# Autodesk Inventor assembly: damascusCoverAssembly
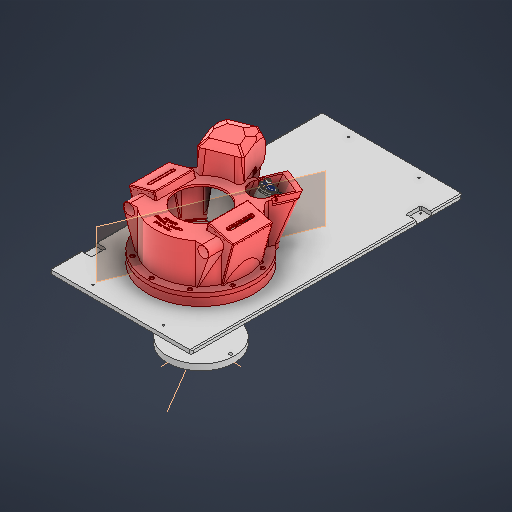
[picture p0: Inventor's stored thumbnail of the model, 512x512]
Saved by Autodesk Inventor 2026.2 (Build 302298000, 298)
## iProperties
Created: 2026-05-01
Part Number: damascusCoverAssembly
Document SubType Name: Assembly
Designer: mayhe
Author: mayhe
## Documents named in this file (10)
- C:\Users\mayhe\OneDrive\Documents\GitHub\In-situ-monitoring-of-powder-bed-fusion-additive-manufacturing\system_development\Damascus\V0.4\hardware development\damascusCoverAssembly.iam
- C:\Users\mayhe\OneDrive\Documents\GitHub\In-situ-monitoring-of-powder-bed-fusion-additive-manufacturing\system_development\Damascus\V0.4\hardware development\Parts\12mm Cover.ipt
- C:\Users\mayhe\OneDrive\Documents\GitHub\In-situ-monitoring-of-powder-bed-fusion-additive-manufacturing\system_development\Damascus\V0.4\hardware development\Parts\Build Plate with 35mm FOV Sketch.ipt
- C:\Users\mayhe\OneDrive\Documents\GitHub\In-situ-monitoring-of-powder-bed-fusion-additive-manufacturing\system_development\Damascus\V0.4\hardware development\Parts\twinHead.ipt
- C:\Users\mayhe\OneDrive\Documents\GitHub\In-situ-monitoring-of-powder-bed-fusion-additive-manufacturing\system_development\Damascus\V0.4\hardware development\Parts\sealRing.ipt
- C:\Users\mayhe\OneDrive\Documents\GitHub\In-situ-monitoring-of-powder-bed-fusion-additive-manufacturing\system_development\Damascus\V0.4\hardware development\Parts\Xi-410-Camera-with-29°-x-18°-Lens\Xi 410 Camera with 29° x.iam
- C:\Users\mayhe\OneDrive\Documents\GitHub\In-situ-monitoring-of-powder-bed-fusion-additive-manufacturing\system_development\Damascus\V0.4\hardware development\Parts\Optical Camera\Camera with 35mm.iam
- C:\Users\mayhe\OneDrive\Documents\GitHub\In-situ-monitoring-of-powder-bed-fusion-additive-manufacturing\system_development\Damascus\V0.4\hardware development\Parts\New Thermal Lid.ipt
- C:\Users\mayhe\OneDrive\Documents\GitHub\In-situ-monitoring-of-powder-bed-fusion-additive-manufacturing\system_development\Damascus\V0.4\hardware development\Parts\Antireflective Glass.ipt
- C:\Users\mayhe\OneDrive\Documents\GitHub\In-situ-monitoring-of-powder-bed-fusion-additive-manufacturing\system_development\Damascus\V0.4\hardware development\Parts\opticalLid.ipt
## Components (9 placed, 9 different names)
1. 12mm Cover:1 — Rotational:1, Rotational:2
2. Build Plate with 35mm FOV Sketch:1 — Rotational:1
3. twinHead:1 — Rotational:3, Mate:3, Mate:4, Mate:5, Mate:6, Rotational:8, Mate:7, Mate:8, Mate:9, Mate:10, Rotational:9
4. sealRing:1 — Rotational:2, Rotational:3, Rotational:5
5. Xi 410 Camera with 29° x:1 [sub-assembly] — Rotational:9
6. Camera with 35mm:1 [sub-assembly] — Rotational:8
7. New Thermal Lid:1 — Mate:3, Mate:4, Mate:9, Mate:10
8. Antireflective Glass:1 — Rotational:5
9. opticalLid:1 — Mate:5, Mate:6, Mate:7, Mate:8
## Relationships (14: Mate 8, RevoluteJoint 6)
- Rotational:1 [RevoluteJoint] (-150 mm): 12mm Cover:1 ↔ Build Plate with 35mm FOV Sketch:1
- Rotational:2 [RevoluteJoint]: 12mm Cover:1 ↔ sealRing:1
- Rotational:3 [RevoluteJoint]: twinHead:1 ↔ sealRing:1
- Mate:3: twinHead:1 ↔ New Thermal Lid:1
- Mate:4: twinHead:1 ↔ New Thermal Lid:1
- Rotational:5 [RevoluteJoint]: sealRing:1 ↔ Antireflective Glass:1
- Mate:5: twinHead:1 ↔ opticalLid:1
- Mate:6: twinHead:1 ↔ opticalLid:1
- Rotational:8 [RevoluteJoint]: twinHead:1 ↔ Camera with 35mm:1
- Mate:7: twinHead:1 ↔ opticalLid:1
- Mate:8: twinHead:1 ↔ opticalLid:1
- Mate:9: twinHead:1 ↔ New Thermal Lid:1
- Mate:10: twinHead:1 ↔ New Thermal Lid:1
- Rotational:9 [RevoluteJoint]: twinHead:1 ↔ Xi 410 Camera with 29° x:1
